# Autodesk Inventor assembly: ensamble caja motriz 2
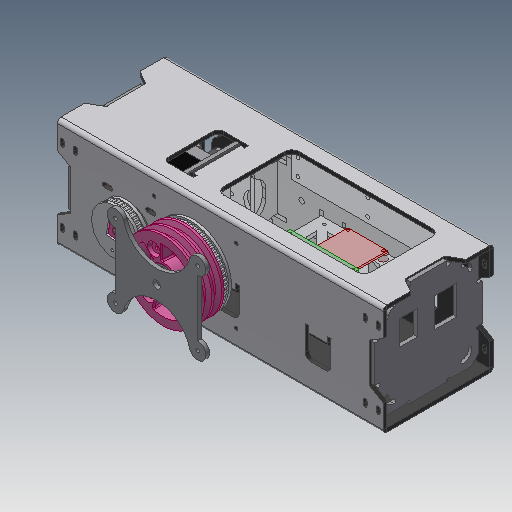
[picture p0: Inventor's stored thumbnail of the model, 512x512]
Saved by Autodesk Inventor 2020 (Build 240168000, 168)
## iProperties
Part Number: ensamble caja motriz 2
Material: Genérico
Document SubType Name: Assembly
Designer: leo
Author: FABLAB
## Documents named in this file (5)
- C:\Users\leo.DESKTOP-592E5E6\Documents\GitHub\TallerDix2022\cad\Inventor\Caja motriz BASE.iam
- C:\Users\leo.DESKTOP-592E5E6\Documents\GitHub\TallerDix2022\cad\Inventor\Caja\componentes.iam
- C:\Users\leo.DESKTOP-592E5E6\Documents\GitHub\TallerDix2022\cad\Inventor\Caja\Case\Case-D.iam
- C:\Users\leo.DESKTOP-592E5E6\Documents\GitHub\TallerDix2022\cad\Inventor\Caja\partes transmision\conjunto polea plato-carrete.iam
- C:\Users\leo.DESKTOP-592E5E6\Documents\GitHub\TallerDix2022\cad\Inventor\Caja\Potencia2.iam
## Components (4 placed, 4 different names)
1. Case-D:1 [sub-assembly] — Coincidencia:1, Coincidencia:4, Nivelación:12, Coincidencia:11, Nivelación:13
2. Potencia2:1 [sub-assembly] — Coincidencia:1, Coincidencia:2, Coincidencia:3
3. conjunto polea plato-carrete:1 [sub-assembly] — Coincidencia:4, Coincidencia:5, Coincidencia:6
4. componentes:1 [sub-assembly] — Nivelación:12, Coincidencia:11, Nivelación:13
## Relationships (9: Mate 7, Flush 2)
- Coincidencia:1 [Mate]: Case-D:1 ↔ Potencia2:1
- Coincidencia:2 [Mate]: Potencia2:1
- Coincidencia:3 [Mate]: Potencia2:1
- Coincidencia:4 [Mate] (5 mm): Case-D:1 ↔ conjunto polea plato-carrete:1
- Coincidencia:5 [Mate]: conjunto polea plato-carrete:1
- Coincidencia:6 [Mate] (72 mm): conjunto polea plato-carrete:1
- Nivelación:12 [Flush]: Case-D:1 ↔ componentes:1
- Coincidencia:11 [Mate]: Case-D:1 ↔ componentes:1
- Nivelación:13 [Flush]: Case-D:1 ↔ componentes:1
